# Autodesk Inventor assembly: 4x2020_subaxis-asm
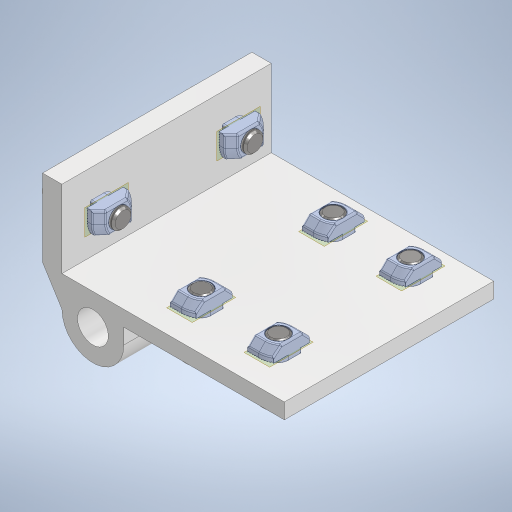
[picture p0: Inventor's stored thumbnail of the model, 512x512]
Saved by Autodesk Inventor 2024 (Build 280153000, 153)
## iProperties
Created: 2025-12-25
Part Number: 4x2020_subaxis-asm
Document SubType Name: Assembly
Designer: schar
Author: schar
## Documents named in this file (7)
- C:\Users\schar\Desktop\projectBlueprint\AMSTS\hardware\4x2020_subaxis-asm.iam
- C:\Users\schar\Desktop\projectBlueprint\AMSTS\hardware\4x2020_subaxis.ipt
- C:\Users\schar\Documents\Inventor\Content Center Files\R2024\en-US\DIN 9021\DIN 9021 - 5,3.ipt
- C:\Users\schar\Desktop\projectBlueprint\AMSTS\hardware\tnut_m5_2020.ipt
- C:\Users\schar\Documents\Inventor\Content Center Files\R2024\en-US\ISO 4762(1)\DIN EN ISO 4762 - M5 x 10.ipt
- C:\Users\schar\Documents\Inventor\Content Center Files\R2024\en-US\ISO 4762(1)\DIN EN ISO 4762 - M5 x 12.ipt
- C:\Users\schar\Documents\Inventor\Content Center Files\R2024\en-US\ISO 4762(1)\DIN EN ISO 4762 - M4 x 8.ipt
## Components (20 placed, 6 different names)
1. 4x2020_subaxis:1 — Mate:1, Mate:2, Mate:3, Mate:4, Mate:7, Mate:8, Mate:9, Mate:10, Mate:24, Mate:25, Mate:26, Mate:27, Mate:28, Mate:29, Mate:32, Rigid:1, Rigid:2, Rigid:3, Rotational:1, Rotational:2, Rotational:3
2. DIN 9021 5,3:1 — Mate:2, Mate:9, Mate:13, Mate:21
3. DIN 9021 5,3:2 — Mate:1, Mate:7, Mate:12, Mate:17
4. DIN 9021 5,3:3 — Mate:3, Mate:10, Mate:14, Mate:20
5. DIN 9021 5,3:4 — Mate:4, Mate:8, Mate:11, Mate:19
6. DIN EN ISO 4762 M5 x 10:2 — Mate:12, Mate:17
7. DIN EN ISO 4762 M5 x 10:3 — Mate:11, Mate:19
8. DIN EN ISO 4762 M5 x 10:4 — Mate:13, Mate:21
9. DIN EN ISO 4762 M5 x 10:5 — Mate:14, Mate:20
10. DIN EN ISO 4762 M4 x 8:1 — Mate:24, Mate:29
11. DIN 9021 5,3:5 — Mate:25, Mate:28, Mate:31, Mate:33
12. DIN 9021 5,3:6 — Mate:26, Mate:27, Mate:30
13. DIN EN ISO 4762 M5 x 12:1 — Mate:31, Mate:33
14. DIN EN ISO 4762 M5 x 12:2 — Mate:30, Mate:32
15. tnut_m5_2020:1 — Rotational:2
16. tnut_m5_2020:2 — Rotational:3
17. tnut_m5_2020:3 — Rigid:3
18. tnut_m5_2020:4 — Rigid:1
19. tnut_m5_2020:5 — Rotational:1
20. tnut_m5_2020:6 — Rigid:2
## Relationships (32: Mate 26, WeldJoint 3, RevoluteJoint 3)
- Mate:1: 4x2020_subaxis:1 ↔ DIN 9021 5,3:2
- Mate:2: 4x2020_subaxis:1 ↔ DIN 9021 5,3:1
- Mate:3: 4x2020_subaxis:1 ↔ DIN 9021 5,3:3
- Mate:4: 4x2020_subaxis:1 ↔ DIN 9021 5,3:4
- Mate:7: 4x2020_subaxis:1 ↔ DIN 9021 5,3:2
- Mate:8: 4x2020_subaxis:1 ↔ DIN 9021 5,3:4
- Mate:9: 4x2020_subaxis:1 ↔ DIN 9021 5,3:1
- Mate:10: 4x2020_subaxis:1 ↔ DIN 9021 5,3:3
- Mate:11: DIN 9021 5,3:4 ↔ DIN EN ISO 4762 M5 x 10:3
- Mate:12: DIN 9021 5,3:2 ↔ DIN EN ISO 4762 M5 x 10:2
- Mate:13: DIN 9021 5,3:1 ↔ DIN EN ISO 4762 M5 x 10:4
- Mate:14: DIN 9021 5,3:3 ↔ DIN EN ISO 4762 M5 x 10:5
- Mate:17: DIN 9021 5,3:2 ↔ DIN EN ISO 4762 M5 x 10:2
- Mate:19: DIN 9021 5,3:4 ↔ DIN EN ISO 4762 M5 x 10:3
- Mate:20: DIN 9021 5,3:3 ↔ DIN EN ISO 4762 M5 x 10:5
- Mate:21: DIN 9021 5,3:1 ↔ DIN EN ISO 4762 M5 x 10:4
- Mate:24: 4x2020_subaxis:1 ↔ DIN EN ISO 4762 M4 x 8:1
- Mate:25: 4x2020_subaxis:1 ↔ DIN 9021 5,3:5
- Mate:26: 4x2020_subaxis:1 ↔ DIN 9021 5,3:6
- Mate:27: 4x2020_subaxis:1 ↔ DIN 9021 5,3:6
- Mate:28: 4x2020_subaxis:1 ↔ DIN 9021 5,3:5
- Mate:29 (4.5 mm): 4x2020_subaxis:1 ↔ DIN EN ISO 4762 M4 x 8:1
- Mate:30: DIN 9021 5,3:6 ↔ DIN EN ISO 4762 M5 x 12:2
- Mate:31: DIN 9021 5,3:5 ↔ DIN EN ISO 4762 M5 x 12:1
- Mate:32: 4x2020_subaxis:1 ↔ DIN EN ISO 4762 M5 x 12:2
- Mate:33: DIN 9021 5,3:5 ↔ DIN EN ISO 4762 M5 x 12:1
- Rigid:1 [WeldJoint] (-0.159 mm): 4x2020_subaxis:1 ↔ tnut_m5_2020:4
- Rigid:2 [WeldJoint] (-0.159 mm): 4x2020_subaxis:1 ↔ tnut_m5_2020:6
- Rigid:3 [WeldJoint] (-0.159 mm): 4x2020_subaxis:1 ↔ tnut_m5_2020:3
- Rotational:1 [RevoluteJoint] (-0.159 mm): 4x2020_subaxis:1 ↔ tnut_m5_2020:5
- Rotational:2 [RevoluteJoint] (-0.159 mm): 4x2020_subaxis:1 ↔ tnut_m5_2020:1
- Rotational:3 [RevoluteJoint] (-0.159 mm): 4x2020_subaxis:1 ↔ tnut_m5_2020:2
